# Autodesk Inventor assembly: mirror render
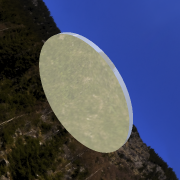
[picture p0: Inventor's stored thumbnail of the model, 180x180]
Saved by Autodesk Inventor 2020 (Build 240168000, 168)
## iProperties
Created: 2024-09-08
Part Number: mirror render
Document SubType Name: Assembly
Designer: 4s
Author: 4s
## Documents named in this file (2)
- C:\Users\4s\Documents\Inventor models\Asterisk\robot_v2\mirror render.iam
- C:\Users\4s\Documents\Inventor models\Asterisk\robot_v2\mirror_50.ipt
## Components (1 placed, 1 different names)
1. mirror_50:2 — Совмещение:1
## Relationships (1: Mate 1)
- Совмещение:1 [Mate] (30 mm): mirror_50:2
